# Autodesk Inventor assembly: Big Drill Complete
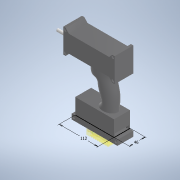
[picture p0: Inventor's stored thumbnail of the model, 180x180]
Saved by Autodesk Inventor 2022 (Build 260153000, 153)
## iProperties
Created: 2021-06-10
Part Number: Big Drill Complete
Document SubType Name: Assembly
Designer: jrcol
Author: jrcol
## Documents named in this file (7)
- C:\Users\jrcol\Desktop\Solar-Lab-Files\Smart Drill\Big Drill Complete.iam
- C:\Users\jrcol\Desktop\Solar-Lab-Files\Smart Drill\Big Housing C.ipt
- C:\Users\jrcol\Desktop\Solar-Lab-Files\Smart Drill\Battery.ipt
- C:\Users\jrcol\Desktop\Solar-Lab-Files\Smart Drill\Big Socket Extension.ipt
- C:\Users\jrcol\Desktop\Solar-Lab-Files\Smart Drill\Micro-Controller.ipt
- C:\Users\jrcol\Desktop\Solar-Lab-Files\Smart Drill\Big Motor.ipt
- C:\Users\jrcol\Desktop\Solar-Lab-Files\Smart Drill\Big shaft coupling.ipt
## Components (6 placed, 6 different names)
1. Big Motor:1
2. Big shaft coupling:1
3. Big Socket Extension:2
4. Big Housing C:1 — Mate:5, Mate:6, Mate:7, Mate:8
5. Battery:1 — Mate:8
6. Micro-Controller:1 — Mate:5, Mate:6, Mate:7
## Relationships (9: Mate 9)
- [Mate]: Big shaft coupling:1 ↔ Big Socket Extension:2
- [Mate] (20 mm): Big Motor:1 ↔ Big Housing C:1
- Mate:5: Big Housing C:1 ↔ Micro-Controller:1
- Mate:6 (-33.5 mm): Big Housing C:1 ↔ Micro-Controller:1
- Mate:7 (-7 mm): Big Housing C:1 ↔ Micro-Controller:1
- Mate:8: Big Housing C:1 ↔ Battery:1
- [Mate]: Big Motor:1 ↔ Big shaft coupling:1
- [Mate]: Big Motor:1 ↔ Big shaft coupling:1
- [Mate]: Big Motor:1 ↔ Big shaft coupling:1
## Named parameters: d33_d1 = 0 mm
